# Autodesk Inventor assembly: Maquina3
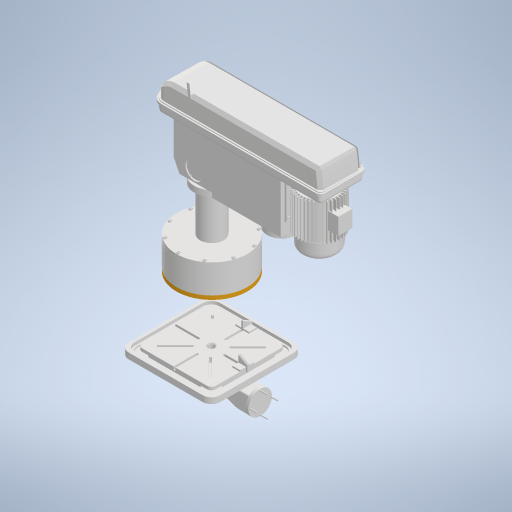
[picture p0: Inventor's stored thumbnail of the model, 512x512]
Saved by Autodesk Inventor 2024.2 (Build 282272000, 272)
## iProperties
Created: 2021-09-13
Part Number: Maquina3
Description: STEP AP203
Document SubType Name: Assembly
Designer: 062210026
Sending System: SolidWorks 2018
Preprocessor: SwSTEP 2.0
Title: multi-spindle.STEP
Author: Moghimi
Revision Number: ANY
## Documents named in this file (20)
- Z:\22AbrV4_ProjInt3\Maquina\Maquina3.iam
- Z:\22AbrV4_ProjInt3\Maquina\maquina\4_Varsay_lan.ipt
- Z:\22AbrV4_ProjInt3\Maquina\maquina\7_Varsay_lan.ipt
- Z:\22AbrV4_ProjInt3\Maquina\maquina\10_Varsay_lan.ipt
- Z:\22AbrV4_ProjInt3\Maquina\maquina\11_Varsay_lan.ipt
- Z:\22AbrV4_ProjInt3\Maquina\maquina\12_Varsay_lan.ipt
- Z:\22AbrV4_ProjInt3\Maquina\maquina\15_Varsay_lan.ipt
- Z:\22AbrV4_ProjInt3\Maquina\maquina\hex bolt gradeab_iso_ISO 4014 - M4 x 35 x 14-N.ipt
- Z:\22AbrV4_ProjInt3\Maquina\maquina\hex bolt gradeab_iso_ISO 4014 - M3 x 20 x 12-N.ipt
- Z:\22AbrV4_ProjInt3\Maquina\maquina\SKF_6004.iam
- Z:\22AbrV4_ProjInt3\Maquina\maquina\MAILN AX.ipt
- Z:\22AbrV4_ProjInt3\Maquina\maquina\helical gear_3_am2_Metric - RH Helical gear 2.5M 30T 45HA 20PA 15FW ---30N75H50L35.0R1.ipt
- Z:\22AbrV4_ProjInt3\Maquina\maquina\SHEL.ipt
- Z:\22AbrV4_ProjInt3\Maquina\maquina\socket head cap screw_am_B18.3.1M - 5 x 0.8 x 20 Hex SHCS -- 20NHX.ipt
- Z:\22AbrV4_ProjInt3\Maquina\maquina\STRIGHTER.ipt
- Z:\22AbrV4_ProjInt3\Maquina\maquina\KEY.ipt
- Z:\22AbrV4_ProjInt3\Maquina\maquina\socket head cap screw_am_B18.3.1M - 5 x 0.8 x 30 Hex SHCS -- 22NHX.ipt
- Z:\22AbrV4_ProjInt3\Maquina\maquina\FIXTURE.ipt
- Z:\22AbrV4_ProjInt3\Tampas\TampaBaixo.ipt
- Z:\22AbrV4_ProjInt3\Tampas\Tampa_Superior.ipt
## Components (55 placed, 46 different names)
1. Tampa_Superior:1 — Mate:12, Mate:13, Mate:14, Mate:15, Mate:16, Mate:17, Mate:18, Mate:19, Mate:20, Mate:21, Mate:22, Mate:23, Mate:24, Mate:25, Mate:26, Mate:27
2. 4_Varsay_lan_3
3. 7_Varsay_lan_6
4. 10_Varsay_lan_9
5. 11_Varsay_lan_10
6. 12_Varsay_lan_11
7. 15_Varsay_lan_16
8. hex bolt gradeab_iso_ISO 4014 - M4 x 35 x 14-N_19
9. hex bolt gradeab_iso_ISO 4014 - M4 x 35 x 14-N_20
10. hex bolt gradeab_iso_ISO 4014 - M4 x 35 x 14-N_21
11. hex bolt gradeab_iso_ISO 4014 - M4 x 35 x 14-N_22
12. hex bolt gradeab_iso_ISO 4014 - M3 x 20 x 12-N_23
13. hex bolt gradeab_iso_ISO 4014 - M3 x 20 x 12-N_24
14. hex bolt gradeab_iso_ISO 4014 - M3 x 20 x 12-N_25
15. hex bolt gradeab_iso_ISO 4014 - M3 x 20 x 12-N_26
16. SKF_6004_34 [sub-assembly]
17. SKF_6004_35 [sub-assembly] — Mate:1
18. MAILN AX_36
19. SKF_6004_39 [sub-assembly]
20. helical gear_3_am2_Metric - RH Helical gear 2.5M 30T 45HA 20PA 15FW ---30N75H50L35.0R1_40
21. SHEL_43 — Mate:12
22. socket head cap screw_am_B18.3.1M - 5 x 0.8 x 20 Hex SHCS -- 20NHX_44 — Mate:13, Mate:14
23. STRIGHTER_46
24. KEY_47
25. SKF_6004_52 [sub-assembly]
26. SKF_6004_53 [sub-assembly]
27. socket head cap screw_am_B18.3.1M - 5 x 0.8 x 20 Hex SHCS -- 20NHX_70
28. socket head cap screw_am_B18.3.1M - 5 x 0.8 x 20 Hex SHCS -- 20NHX_71 — Mate:25, Mate:26, Mate:27
29. socket head cap screw_am_B18.3.1M - 5 x 0.8 x 20 Hex SHCS -- 20NHX_72 — Mate:23, Mate:24
30. socket head cap screw_am_B18.3.1M - 5 x 0.8 x 20 Hex SHCS -- 20NHX_73 — Mate:21, Mate:22
31. socket head cap screw_am_B18.3.1M - 5 x 0.8 x 20 Hex SHCS -- 20NHX_75 — Mate:19, Mate:20
32. socket head cap screw_am_B18.3.1M - 5 x 0.8 x 20 Hex SHCS -- 20NHX_76 — Mate:17, Mate:18
33. socket head cap screw_am_B18.3.1M - 5 x 0.8 x 20 Hex SHCS -- 20NHX_77 — Mate:15, Mate:16
34. socket head cap screw_am_B18.3.1M - 5 x 0.8 x 20 Hex SHCS -- 20NHX_78
35. socket head cap screw_am_B18.3.1M - 5 x 0.8 x 30 Hex SHCS -- 22NHX_98
36. socket head cap screw_am_B18.3.1M - 5 x 0.8 x 30 Hex SHCS -- 22NHX_99
37. socket head cap screw_am_B18.3.1M - 5 x 0.8 x 30 Hex SHCS -- 22NHX_100
38. socket head cap screw_am_B18.3.1M - 5 x 0.8 x 30 Hex SHCS -- 22NHX_101
39. socket head cap screw_am_B18.3.1M - 5 x 0.8 x 30 Hex SHCS -- 22NHX_102
40. socket head cap screw_am_B18.3.1M - 5 x 0.8 x 30 Hex SHCS -- 22NHX_103
41. socket head cap screw_am_B18.3.1M - 5 x 0.8 x 30 Hex SHCS -- 22NHX_104
42. FIXTURE_111
43. FIXTURE_112
44. TampaBaixo:1 — Mate:1, Mate:3, Mate:4, Mate:5, Mate:6, Mate:7, Mate:8, Mate:9, Mate:10, Mate:11
45. socket head cap screw_am_B18.3.1M - 5 x 0.8 x 20 Hex SHCS -- 20NHX:21 — Mate:3
46. socket head cap screw_am_B18.3.1M - 5 x 0.8 x 20 Hex SHCS -- 20NHX:22 — Mate:8
47. socket head cap screw_am_B18.3.1M - 5 x 0.8 x 20 Hex SHCS -- 20NHX:23 — Mate:10
48. socket head cap screw_am_B18.3.1M - 5 x 0.8 x 20 Hex SHCS -- 20NHX:24
49. socket head cap screw_am_B18.3.1M - 5 x 0.8 x 20 Hex SHCS -- 20NHX:26 — Mate:5
50. socket head cap screw_am_B18.3.1M - 5 x 0.8 x 20 Hex SHCS -- 20NHX:27 — Mate:6
51. socket head cap screw_am_B18.3.1M - 5 x 0.8 x 20 Hex SHCS -- 20NHX:28 — Mate:9
52. socket head cap screw_am_B18.3.1M - 5 x 0.8 x 20 Hex SHCS -- 20NHX:30 — Mate:11
53. socket head cap screw_am_B18.3.1M - 5 x 0.8 x 20 Hex SHCS -- 20NHX:32 — Mate:7
54. socket head cap screw_am_B18.3.1M - 5 x 0.8 x 20 Hex SHCS -- 20NHX:33 — Mate:4
55. socket head cap screw_am_B18.3.1M - 5 x 0.8 x 20 Hex SHCS -- 20NHX_74
## Relationships (26: Mate 26)
- Mate:1: SKF_6004_35 ↔ TampaBaixo:1
- Mate:3: TampaBaixo:1 ↔ socket head cap screw_am_B18.3.1M - 5 x 0.8 x 20 Hex SHCS -- 20NHX:21
- Mate:4: TampaBaixo:1 ↔ socket head cap screw_am_B18.3.1M - 5 x 0.8 x 20 Hex SHCS -- 20NHX:33
- Mate:5: TampaBaixo:1 ↔ socket head cap screw_am_B18.3.1M - 5 x 0.8 x 20 Hex SHCS -- 20NHX:26
- Mate:6: TampaBaixo:1 ↔ socket head cap screw_am_B18.3.1M - 5 x 0.8 x 20 Hex SHCS -- 20NHX:27
- Mate:7: TampaBaixo:1 ↔ socket head cap screw_am_B18.3.1M - 5 x 0.8 x 20 Hex SHCS -- 20NHX:32
- Mate:8: TampaBaixo:1 ↔ socket head cap screw_am_B18.3.1M - 5 x 0.8 x 20 Hex SHCS -- 20NHX:22
- Mate:9: TampaBaixo:1 ↔ socket head cap screw_am_B18.3.1M - 5 x 0.8 x 20 Hex SHCS -- 20NHX:28
- Mate:10: TampaBaixo:1 ↔ socket head cap screw_am_B18.3.1M - 5 x 0.8 x 20 Hex SHCS -- 20NHX:23
- Mate:11: TampaBaixo:1 ↔ socket head cap screw_am_B18.3.1M - 5 x 0.8 x 20 Hex SHCS -- 20NHX:30
- Mate:12: Tampa_Superior:1 ↔ SHEL_43
- Mate:13: Tampa_Superior:1 ↔ socket head cap screw_am_B18.3.1M - 5 x 0.8 x 20 Hex SHCS -- 20NHX_44
- Mate:14: Tampa_Superior:1 ↔ socket head cap screw_am_B18.3.1M - 5 x 0.8 x 20 Hex SHCS -- 20NHX_44
- Mate:15: Tampa_Superior:1 ↔ socket head cap screw_am_B18.3.1M - 5 x 0.8 x 20 Hex SHCS -- 20NHX_77
- Mate:16: Tampa_Superior:1 ↔ socket head cap screw_am_B18.3.1M - 5 x 0.8 x 20 Hex SHCS -- 20NHX_77
- Mate:17: Tampa_Superior:1 ↔ socket head cap screw_am_B18.3.1M - 5 x 0.8 x 20 Hex SHCS -- 20NHX_76
- Mate:18: Tampa_Superior:1 ↔ socket head cap screw_am_B18.3.1M - 5 x 0.8 x 20 Hex SHCS -- 20NHX_76
- Mate:19: Tampa_Superior:1 ↔ socket head cap screw_am_B18.3.1M - 5 x 0.8 x 20 Hex SHCS -- 20NHX_75
- Mate:20: Tampa_Superior:1 ↔ socket head cap screw_am_B18.3.1M - 5 x 0.8 x 20 Hex SHCS -- 20NHX_75
- Mate:21: Tampa_Superior:1 ↔ socket head cap screw_am_B18.3.1M - 5 x 0.8 x 20 Hex SHCS -- 20NHX_73
- Mate:22: Tampa_Superior:1 ↔ socket head cap screw_am_B18.3.1M - 5 x 0.8 x 20 Hex SHCS -- 20NHX_73
- Mate:23: Tampa_Superior:1 ↔ socket head cap screw_am_B18.3.1M - 5 x 0.8 x 20 Hex SHCS -- 20NHX_72
- Mate:24: Tampa_Superior:1 ↔ socket head cap screw_am_B18.3.1M - 5 x 0.8 x 20 Hex SHCS -- 20NHX_72
- Mate:25: Tampa_Superior:1 ↔ socket head cap screw_am_B18.3.1M - 5 x 0.8 x 20 Hex SHCS -- 20NHX_71
- Mate:26: Tampa_Superior:1 ↔ socket head cap screw_am_B18.3.1M - 5 x 0.8 x 20 Hex SHCS -- 20NHX_71
- Mate:27: Tampa_Superior:1 ↔ socket head cap screw_am_B18.3.1M - 5 x 0.8 x 20 Hex SHCS -- 20NHX_71
